(part 1 of 2)
# Autodesk Inventor assembly: ODrive Pro Assembly
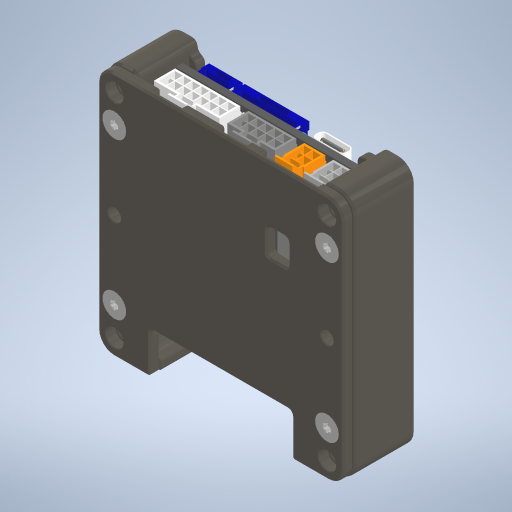
[picture p0: Inventor's stored thumbnail of the model, 512x512]
Saved by Autodesk Inventor 2023.4 (Build 274418000, 418)
## iProperties
Created: 2025-03-02
Part Number: ODrive Pro Assembly
Description: STEP AP242
Document SubType Name: Assembly
Designer: aaron
Title: 67c5018548154165ea0d0b83
Sending System: ONSHAPE BY PTC INC, 1.194
Preprocessor: ST-DEVELOPER v20
## Documents named in this file (723)
- C:\work\openworkout\digital_weight_device\cad\v5\odrive\ODrive Pro Assembly\ODrive Pro Assembly.iam
- C:\work\openworkout\digital_weight_device\cad\v5\odrive\ODrive Pro Assembly\92703A148_18-8 Stainless Steel Torx Flat Head Screws.ipt
- C:\work\openworkout\digital_weight_device\cad\v5\odrive\ODrive Pro Assembly\___________10 SIZE CODE G_7.ipt
- C:\work\openworkout\digital_weight_device\cad\v5\odrive\ODrive Pro Assembly\SOT23-5.ipt
- C:\work\openworkout\digital_weight_device\cad\v5\odrive\ODrive Pro Assembly\Extruded_55.ipt
- C:\work\openworkout\digital_weight_device\cad\v5\odrive\ODrive Pro Assembly\Open CASCADE STEP translator 6.8 23.2.1_6.ipt
- C:\work\openworkout\digital_weight_device\cad\v5\odrive\ODrive Pro Assembly\Extruded_11.ipt
- C:\work\openworkout\digital_weight_device\cad\v5\odrive\ODrive Pro Assembly\Extruded_52.ipt
- C:\work\openworkout\digital_weight_device\cad\v5\odrive\ODrive Pro Assembly\Extruded.ipt
- C:\work\openworkout\digital_weight_device\cad\v5\odrive\ODrive Pro Assembly\________10 SIZE CODE G_1.ipt
- C:\work\openworkout\digital_weight_device\cad\v5\odrive\ODrive Pro Assembly\Leader_24.ipt
- C:\work\openworkout\digital_weight_device\cad\v5\odrive\ODrive Pro Assembly\Extruded_19.ipt
- C:\work\openworkout\digital_weight_device\cad\v5\odrive\ODrive Pro Assembly\Open CASCADE STEP translator 6.8 23.2.1_2.ipt
- C:\work\openworkout\digital_weight_device\cad\v5\odrive\ODrive Pro Assembly\Open CASCADE STEP translator 6.8 23.2.1_2_1.ipt
- C:\work\openworkout\digital_weight_device\cad\v5\odrive\ODrive Pro Assembly\Extruded_16.ipt
- C:\work\openworkout\digital_weight_device\cad\v5\odrive\ODrive Pro Assembly\Cylinder_18.ipt
- C:\work\openworkout\digital_weight_device\cad\v5\odrive\ODrive Pro Assembly\Extruded_13.ipt
- C:\work\openworkout\digital_weight_device\cad\v5\odrive\ODrive Pro Assembly\Extruded_35.ipt
- C:\work\openworkout\digital_weight_device\cad\v5\odrive\ODrive Pro Assembly\Extruded_24.ipt
- C:\work\openworkout\digital_weight_device\cad\v5\odrive\ODrive Pro Assembly\Mid_Body_3.ipt
- C:\work\openworkout\digital_weight_device\cad\v5\odrive\ODrive Pro Assembly\Open CASCADE STEP translator 6.8 2.1.2.ipt
- C:\work\openworkout\digital_weight_device\cad\v5\odrive\ODrive Pro Assembly\RES 0603 (1608 metric)_21.ipt
- C:\work\openworkout\digital_weight_device\cad\v5\odrive\ODrive Pro Assembly\Extruded_10.ipt
- C:\work\openworkout\digital_weight_device\cad\v5\odrive\ODrive Pro Assembly\Extruded_42.ipt
- C:\work\openworkout\digital_weight_device\cad\v5\odrive\ODrive Pro Assembly\Leader_1.ipt
- C:\work\openworkout\digital_weight_device\cad\v5\odrive\ODrive Pro Assembly\Open CASCADE STEP translator 6.8 26.4.1_6.ipt
- C:\work\openworkout\digital_weight_device\cad\v5\odrive\ODrive Pro Assembly\Open CASCADE STEP translator 6.8 18.2.1.ipt
- C:\work\openworkout\digital_weight_device\cad\v5\odrive\ODrive Pro Assembly\FDMS86300DC rev A_7.ipt
- C:\work\openworkout\digital_weight_device\cad\v5\odrive\ODrive Pro Assembly\Extruded_21.ipt
- C:\work\openworkout\digital_weight_device\cad\v5\odrive\ODrive Pro Assembly\Mid_Body_1.ipt
- C:\work\openworkout\digital_weight_device\cad\v5\odrive\ODrive Pro Assembly\Extruded_31.ipt
- C:\work\openworkout\digital_weight_device\cad\v5\odrive\ODrive Pro Assembly\Extruded_6.ipt
- C:\work\openworkout\digital_weight_device\cad\v5\odrive\ODrive Pro Assembly\Extruded_34.ipt
- C:\work\openworkout\digital_weight_device\cad\v5\odrive\ODrive Pro Assembly\Cylinder_3.ipt
- C:\work\openworkout\digital_weight_device\cad\v5\odrive\ODrive Pro Assembly\Extruded_16_1.ipt
- C:\work\openworkout\digital_weight_device\cad\v5\odrive\ODrive Pro Assembly\Extruded_26.ipt
- C:\work\openworkout\digital_weight_device\cad\v5\odrive\ODrive Pro Assembly\Open CASCADE STEP translator 6.8 23.2.1_4.ipt
- C:\work\openworkout\digital_weight_device\cad\v5\odrive\ODrive Pro Assembly\Extruded_37.ipt
- C:\work\openworkout\digital_weight_device\cad\v5\odrive\ODrive Pro Assembly\Mark_4.ipt
- C:\work\openworkout\digital_weight_device\cad\v5\odrive\ODrive Pro Assembly\Open CASCADE STEP translator 6.8 23.2.1_11.ipt
- C:\work\openworkout\digital_weight_device\cad\v5\odrive\ODrive Pro Assembly\Mark.ipt
- C:\work\openworkout\digital_weight_device\cad\v5\odrive\ODrive Pro Assembly\Extruded_10_1.ipt
- C:\work\openworkout\digital_weight_device\cad\v5\odrive\ODrive Pro Assembly\Extruded_31_1.ipt
- C:\work\openworkout\digital_weight_device\cad\v5\odrive\ODrive Pro Assembly\Extruded_63.ipt
- C:\work\openworkout\digital_weight_device\cad\v5\odrive\ODrive Pro Assembly\Extruded_35_1.ipt
- C:\work\openworkout\digital_weight_device\cad\v5\odrive\ODrive Pro Assembly\Extruded_38.ipt
- C:\work\openworkout\digital_weight_device\cad\v5\odrive\ODrive Pro Assembly\Open CASCADE STEP translator 6.8 26.1.ipt
- C:\work\openworkout\digital_weight_device\cad\v5\odrive\ODrive Pro Assembly\Extruded_17.ipt
- C:\work\openworkout\digital_weight_device\cad\v5\odrive\ODrive Pro Assembly\Extruded_7.ipt
- C:\work\openworkout\digital_weight_device\cad\v5\odrive\ODrive Pro Assembly\Extruded_2.ipt
- C:\work\openworkout\digital_weight_device\cad\v5\odrive\ODrive Pro Assembly\Open CASCADE STEP translator 6.8 43.4.1_6.ipt
- C:\work\openworkout\digital_weight_device\cad\v5\odrive\ODrive Pro Assembly\Extruded_1.ipt
- C:\work\openworkout\digital_weight_device\cad\v5\odrive\ODrive Pro Assembly\Extruded_13_1.ipt
- C:\work\openworkout\digital_weight_device\cad\v5\odrive\ODrive Pro Assembly\Cylinder_8.ipt
- C:\work\openworkout\digital_weight_device\cad\v5\odrive\ODrive Pro Assembly\Extruded_3.ipt
- C:\work\openworkout\digital_weight_device\cad\v5\odrive\ODrive Pro Assembly\Open CASCADE STEP translator 6.8 2.1.1.ipt
- C:\work\openworkout\digital_weight_device\cad\v5\odrive\ODrive Pro Assembly\Extruded_4.ipt
- C:\work\openworkout\digital_weight_device\cad\v5\odrive\ODrive Pro Assembly\Extruded_10_2.ipt
- C:\work\openworkout\digital_weight_device\cad\v5\odrive\ODrive Pro Assembly\lead.ipt
- C:\work\openworkout\digital_weight_device\cad\v5\odrive\ODrive Pro Assembly\___________10 SIZE CODE G_4.ipt
- C:\work\openworkout\digital_weight_device\cad\v5\odrive\ODrive Pro Assembly\Extruded_2_1.ipt
- C:\work\openworkout\digital_weight_device\cad\v5\odrive\ODrive Pro Assembly\Mid_Body_3_1.ipt
- C:\work\openworkout\digital_weight_device\cad\v5\odrive\ODrive Pro Assembly\Extruded_23.ipt
- C:\work\openworkout\digital_weight_device\cad\v5\odrive\ODrive Pro Assembly\bottom.ipt
- C:\work\openworkout\digital_weight_device\cad\v5\odrive\ODrive Pro Assembly\Open CASCADE STEP translator 6.8 23.2.1_3.ipt
- C:\work\openworkout\digital_weight_device\cad\v5\odrive\ODrive Pro Assembly\Extruded_5.ipt
- C:\work\openworkout\digital_weight_device\cad\v5\odrive\ODrive Pro Assembly\NONE.ipt
- C:\work\openworkout\digital_weight_device\cad\v5\odrive\ODrive Pro Assembly\Extruded_2_2.ipt
- C:\work\openworkout\digital_weight_device\cad\v5\odrive\ODrive Pro Assembly\Open CASCADE STEP translator 6.8 2.1.1_1.ipt
- C:\work\openworkout\digital_weight_device\cad\v5\odrive\ODrive Pro Assembly\Extruded_6_1.ipt
- C:\work\openworkout\digital_weight_device\cad\v5\odrive\ODrive Pro Assembly\Mark_1.ipt
- C:\work\openworkout\digital_weight_device\cad\v5\odrive\ODrive Pro Assembly\Extruded_1_1.ipt
- C:\work\openworkout\digital_weight_device\cad\v5\odrive\ODrive Pro Assembly\Open CASCADE STEP translator 6.8 43.1.ipt
- C:\work\openworkout\digital_weight_device\cad\v5\odrive\ODrive Pro Assembly\Leader_17.ipt
- C:\work\openworkout\digital_weight_device\cad\v5\odrive\ODrive Pro Assembly\Open CASCADE STEP translator 6.8 43.4.1_13.ipt
- C:\work\openworkout\digital_weight_device\cad\v5\odrive\ODrive Pro Assembly\Extruded_8.ipt
- C:\work\openworkout\digital_weight_device\cad\v5\odrive\ODrive Pro Assembly\Leader_3.ipt
- C:\work\openworkout\digital_weight_device\cad\v5\odrive\ODrive Pro Assembly\Extruded_2_3.ipt
- C:\work\openworkout\digital_weight_device\cad\v5\odrive\ODrive Pro Assembly\Extruded_11_1.ipt
- C:\work\openworkout\digital_weight_device\cad\v5\odrive\ODrive Pro Assembly\Lead_4.ipt
- C:\work\openworkout\digital_weight_device\cad\v5\odrive\ODrive Pro Assembly\RPC2512_stp.ipt
- C:\work\openworkout\digital_weight_device\cad\v5\odrive\ODrive Pro Assembly\Mid_Body_2.ipt
- C:\work\openworkout\digital_weight_device\cad\v5\odrive\ODrive Pro Assembly\Extruded_3_1.ipt
- C:\work\openworkout\digital_weight_device\cad\v5\odrive\ODrive Pro Assembly\Cylinder_12.ipt
- C:\work\openworkout\digital_weight_device\cad\v5\odrive\ODrive Pro Assembly\Extruded_32.ipt
- C:\work\openworkout\digital_weight_device\cad\v5\odrive\ODrive Pro Assembly\Open CASCADE STEP translator 6.8 2.1.1_1_1.ipt
- C:\work\openworkout\digital_weight_device\cad\v5\odrive\ODrive Pro Assembly\Leader_10.ipt
- C:\work\openworkout\digital_weight_device\cad\v5\odrive\ODrive Pro Assembly\Extruded_9.ipt
- C:\work\openworkout\digital_weight_device\cad\v5\odrive\ODrive Pro Assembly\Open CASCADE STEP translator 7.5 6.74.2.1.ipt
- C:\work\openworkout\digital_weight_device\cad\v5\odrive\ODrive Pro Assembly\Extruded_2_4.ipt
- C:\work\openworkout\digital_weight_device\cad\v5\odrive\ODrive Pro Assembly\Cylinder_16.ipt
- C:\work\openworkout\digital_weight_device\cad\v5\odrive\ODrive Pro Assembly\Extruded_23_1.ipt
- C:\work\openworkout\digital_weight_device\cad\v5\odrive\ODrive Pro Assembly\Extruded_13_2.ipt
- C:\work\openworkout\digital_weight_device\cad\v5\odrive\ODrive Pro Assembly\Extruded_12.ipt
- C:\work\openworkout\digital_weight_device\cad\v5\odrive\ODrive Pro Assembly\________10 SIZE CODE G.ipt
- C:\work\openworkout\digital_weight_device\cad\v5\odrive\ODrive Pro Assembly\Leader_23.ipt
- C:\work\openworkout\digital_weight_device\cad\v5\odrive\ODrive Pro Assembly\Extruded_18.ipt
- C:\work\openworkout\digital_weight_device\cad\v5\odrive\ODrive Pro Assembly\Mid_Body_1_1.ipt
- C:\work\openworkout\digital_weight_device\cad\v5\odrive\ODrive Pro Assembly\Mid_Body_1_2.ipt
- C:\work\openworkout\digital_weight_device\cad\v5\odrive\ODrive Pro Assembly\Extruded_7_1.ipt
- C:\work\openworkout\digital_weight_device\cad\v5\odrive\ODrive Pro Assembly\Extruded_22.ipt
- C:\work\openworkout\digital_weight_device\cad\v5\odrive\ODrive Pro Assembly\Extruded_12_1.ipt
- C:\work\openworkout\digital_weight_device\cad\v5\odrive\ODrive Pro Assembly\Extruded_34_1.ipt
- C:\work\openworkout\digital_weight_device\cad\v5\odrive\ODrive Pro Assembly\Extruded_49.ipt
- C:\work\openworkout\digital_weight_device\cad\v5\odrive\ODrive Pro Assembly\Mark_2.ipt
- C:\work\openworkout\digital_weight_device\cad\v5\odrive\ODrive Pro Assembly\Open CASCADE STEP translator 6.8 2.1.1_2.ipt
- C:\work\openworkout\digital_weight_device\cad\v5\odrive\ODrive Pro Assembly\RES 0603 (1608 metric)_20.ipt
- C:\work\openworkout\digital_weight_device\cad\v5\odrive\ODrive Pro Assembly\Extruded_3_2.ipt
- C:\work\openworkout\digital_weight_device\cad\v5\odrive\ODrive Pro Assembly\Extruded_7_2.ipt
- C:\work\openworkout\digital_weight_device\cad\v5\odrive\ODrive Pro Assembly\Leader.ipt
- C:\work\openworkout\digital_weight_device\cad\v5\odrive\ODrive Pro Assembly\Open CASCADE STEP translator 6.8 26.4.1_5.ipt
- C:\work\openworkout\digital_weight_device\cad\v5\odrive\ODrive Pro Assembly\Mid_Body.ipt
- C:\work\openworkout\digital_weight_device\cad\v5\odrive\ODrive Pro Assembly\FDMS86300DC rev A_6.ipt
- C:\work\openworkout\digital_weight_device\cad\v5\odrive\ODrive Pro Assembly\Extruded_43.ipt
- C:\work\openworkout\digital_weight_device\cad\v5\odrive\ODrive Pro Assembly\Mark_3.ipt
- C:\work\openworkout\digital_weight_device\cad\v5\odrive\ODrive Pro Assembly\Extruded_15.ipt
- C:\work\openworkout\digital_weight_device\cad\v5\odrive\ODrive Pro Assembly\Extruded_13_3.ipt
- C:\work\openworkout\digital_weight_device\cad\v5\odrive\ODrive Pro Assembly\RES 0603 (1608 metric)_11.ipt
- C:\work\openworkout\digital_weight_device\cad\v5\odrive\ODrive Pro Assembly\Cylinder_2.ipt
- C:\work\openworkout\digital_weight_device\cad\v5\odrive\ODrive Pro Assembly\Extruded_33.ipt
- C:\work\openworkout\digital_weight_device\cad\v5\odrive\ODrive Pro Assembly\Extruded_12_2.ipt
- C:\work\openworkout\digital_weight_device\cad\v5\odrive\ODrive Pro Assembly\Mid_Body_2_1.ipt
- C:\work\openworkout\digital_weight_device\cad\v5\odrive\ODrive Pro Assembly\Extruded_36.ipt
- C:\work\openworkout\digital_weight_device\cad\v5\odrive\ODrive Pro Assembly\Extruded_9_1.ipt
- C:\work\openworkout\digital_weight_device\cad\v5\odrive\ODrive Pro Assembly\Open CASCADE STEP translator 6.8 2.1.1_3.ipt
- C:\work\openworkout\digital_weight_device\cad\v5\odrive\ODrive Pro Assembly\______10 SIZE CODE G_2.ipt
- C:\work\openworkout\digital_weight_device\cad\v5\odrive\ODrive Pro Assembly\Extruded_5_1.ipt
- C:\work\openworkout\digital_weight_device\cad\v5\odrive\ODrive Pro Assembly\Extruded_12_3.ipt
- C:\work\openworkout\digital_weight_device\cad\v5\odrive\ODrive Pro Assembly\Open CASCADE STEP translator 6.8 23.2.1_9.ipt
- C:\work\openworkout\digital_weight_device\cad\v5\odrive\ODrive Pro Assembly\Open CASCADE STEP translator 6.8 23.2.1_10.ipt
- C:\work\openworkout\digital_weight_device\cad\v5\odrive\ODrive Pro Assembly\Open CASCADE STEP translator 6.8 1.2.1_1.ipt
- C:\work\openworkout\digital_weight_device\cad\v5\odrive\ODrive Pro Assembly\Extruded_19_1.ipt
- C:\work\openworkout\digital_weight_device\cad\v5\odrive\ODrive Pro Assembly\Extruded_30.ipt
- C:\work\openworkout\digital_weight_device\cad\v5\odrive\ODrive Pro Assembly\Extruded_62.ipt
- C:\work\openworkout\digital_weight_device\cad\v5\odrive\ODrive Pro Assembly\Extruded_34_2.ipt
- C:\work\openworkout\digital_weight_device\cad\v5\odrive\ODrive Pro Assembly\Mark_4_1.ipt
- C:\work\openworkout\digital_weight_device\cad\v5\odrive\ODrive Pro Assembly\Extruded_20.ipt
- C:\work\openworkout\digital_weight_device\cad\v5\odrive\ODrive Pro Assembly\Extruded_16_2.ipt
- C:\work\openworkout\digital_weight_device\cad\v5\odrive\ODrive Pro Assembly\___________10 SIZE CODE G_6.ipt
- C:\work\openworkout\digital_weight_device\cad\v5\odrive\ODrive Pro Assembly\Extruded_12_4.ipt
- C:\work\openworkout\digital_weight_device\cad\v5\odrive\ODrive Pro Assembly\Extruded_54.ipt
- C:\work\openworkout\digital_weight_device\cad\v5\odrive\ODrive Pro Assembly\Mid_Body_3_2.ipt
- C:\work\openworkout\digital_weight_device\cad\v5\odrive\ODrive Pro Assembly\Open CASCADE STEP translator 6.8 43.4.1_5.ipt
- C:\work\openworkout\digital_weight_device\cad\v5\odrive\ODrive Pro Assembly\Extruded_3_3.ipt
- C:\work\openworkout\digital_weight_device\cad\v5\odrive\ODrive Pro Assembly\Extruded_12_5.ipt
- C:\work\openworkout\digital_weight_device\cad\v5\odrive\ODrive Pro Assembly\Cylinder_7.ipt
- C:\work\openworkout\digital_weight_device\cad\v5\odrive\ODrive Pro Assembly\Extruded_1_2.ipt
- C:\work\openworkout\digital_weight_device\cad\v5\odrive\ODrive Pro Assembly\Open CASCADE STEP translator 6.8 19.2.1.ipt
- C:\work\openworkout\digital_weight_device\cad\v5\odrive\ODrive Pro Assembly\Extruded_1_3.ipt
- C:\work\openworkout\digital_weight_device\cad\v5\odrive\ODrive Pro Assembly\Extruded_22_1.ipt
- C:\work\openworkout\digital_weight_device\cad\v5\odrive\ODrive Pro Assembly\top.ipt
- C:\work\openworkout\digital_weight_device\cad\v5\odrive\ODrive Pro Assembly\Open CASCADE STEP translator 6.8 23.2.1_2_2.ipt
- C:\work\openworkout\digital_weight_device\cad\v5\odrive\ODrive Pro Assembly\Extruded_7_3.ipt
- C:\work\openworkout\digital_weight_device\cad\v5\odrive\ODrive Pro Assembly\Cylinder_9.ipt
- C:\work\openworkout\digital_weight_device\cad\v5\odrive\ODrive Pro Assembly\SM05B-GHS-TB.ipt
- C:\work\openworkout\digital_weight_device\cad\v5\odrive\ODrive Pro Assembly\Mark_2_1.ipt
- C:\work\openworkout\digital_weight_device\cad\v5\odrive\ODrive Pro Assembly\Extruded_5_2.ipt
- C:\work\openworkout\digital_weight_device\cad\v5\odrive\ODrive Pro Assembly\Open CASCADE STEP translator 6.8 23.2.1_1.ipt
- C:\work\openworkout\digital_weight_device\cad\v5\odrive\ODrive Pro Assembly\Extruded_14.ipt
- C:\work\openworkout\digital_weight_device\cad\v5\odrive\ODrive Pro Assembly\Extruded_4_1.ipt
- C:\work\openworkout\digital_weight_device\cad\v5\odrive\ODrive Pro Assembly\Leader_16.ipt
- C:\work\openworkout\digital_weight_device\cad\v5\odrive\ODrive Pro Assembly\Open CASCADE STEP translator 6.8 43.4.1_12.ipt
- C:\work\openworkout\digital_weight_device\cad\v5\odrive\ODrive Pro Assembly\Extruded_16_3.ipt
- C:\work\openworkout\digital_weight_device\cad\v5\odrive\ODrive Pro Assembly\Leader_2.ipt
- C:\work\openworkout\digital_weight_device\cad\v5\odrive\ODrive Pro Assembly\Extruded_25.ipt
- C:\work\openworkout\digital_weight_device\cad\v5\odrive\ODrive Pro Assembly\Extruded_5_3.ipt
- C:\work\openworkout\digital_weight_device\cad\v5\odrive\ODrive Pro Assembly\Lead_3.ipt
- C:\work\openworkout\digital_weight_device\cad\v5\odrive\ODrive Pro Assembly\RPC2512_stp_1.ipt
- C:\work\openworkout\digital_weight_device\cad\v5\odrive\ODrive Pro Assembly\Mark_1_1.ipt
- C:\work\openworkout\digital_weight_device\cad\v5\odrive\ODrive Pro Assembly\Extruded_6_2.ipt
- C:\work\openworkout\digital_weight_device\cad\v5\odrive\ODrive Pro Assembly\Cylinder_11.ipt
- C:\work\openworkout\digital_weight_device\cad\v5\odrive\ODrive Pro Assembly\Extruded_15_1.ipt
- C:\work\openworkout\digital_weight_device\cad\v5\odrive\ODrive Pro Assembly\Leader_2_1.ipt
- C:\work\openworkout\digital_weight_device\cad\v5\odrive\ODrive Pro Assembly\Leader_9.ipt
- C:\work\openworkout\digital_weight_device\cad\v5\odrive\ODrive Pro Assembly\Extruded_19_2.ipt
- C:\work\openworkout\digital_weight_device\cad\v5\odrive\ODrive Pro Assembly\Extruded_5_4.ipt
- C:\work\openworkout\digital_weight_device\cad\v5\odrive\ODrive Pro Assembly\Cylinder_15.ipt
- C:\work\openworkout\digital_weight_device\cad\v5\odrive\ODrive Pro Assembly\Extruded_15_2.ipt
- C:\work\openworkout\digital_weight_device\cad\v5\odrive\ODrive Pro Assembly\Extruded_5_5.ipt
- C:\work\openworkout\digital_weight_device\cad\v5\odrive\ODrive Pro Assembly\Leader_22.ipt
- C:\work\openworkout\digital_weight_device\cad\v5\odrive\ODrive Pro Assembly\Extruded_27.ipt
- C:\work\openworkout\digital_weight_device\cad\v5\odrive\ODrive Pro Assembly\Extruded_9_2.ipt
- C:\work\openworkout\digital_weight_device\cad\v5\odrive\ODrive Pro Assembly\Mark_5.ipt
- C:\work\openworkout\digital_weight_device\cad\v5\odrive\ODrive Pro Assembly\Extruded_15_3.ipt
- C:\work\openworkout\digital_weight_device\cad\v5\odrive\ODrive Pro Assembly\Extruded_48.ipt
- C:\work\openworkout\digital_weight_device\cad\v5\odrive\ODrive Pro Assembly\Open CASCADE STEP translator 6.8 2.2.1_2.ipt
- C:\work\openworkout\digital_weight_device\cad\v5\odrive\ODrive Pro Assembly\Extruded_3_4.ipt
- C:\work\openworkout\digital_weight_device\cad\v5\odrive\ODrive Pro Assembly\Open CASCADE STEP translator 6.8 5.2.1.ipt
- C:\work\openworkout\digital_weight_device\cad\v5\odrive\ODrive Pro Assembly\Leader_15.ipt
- C:\work\openworkout\digital_weight_device\cad\v5\odrive\ODrive Pro Assembly\Extruded_42_1.ipt
- C:\work\openworkout\digital_weight_device\cad\v5\odrive\ODrive Pro Assembly\Open CASCADE STEP translator 7.5 6.122.1.1.ipt
- C:\work\openworkout\digital_weight_device\cad\v5\odrive\ODrive Pro Assembly\Extruded_12_6.ipt
- C:\work\openworkout\digital_weight_device\cad\v5\odrive\ODrive Pro Assembly\Cylinder_1.ipt
- C:\work\openworkout\digital_weight_device\cad\v5\odrive\ODrive Pro Assembly\Extruded_25_1.ipt
- C:\work\openworkout\digital_weight_device\cad\v5\odrive\ODrive Pro Assembly\Extruded_17_1.ipt
- C:\work\openworkout\digital_weight_device\cad\v5\odrive\ODrive Pro Assembly\Extruded_4_2.ipt
- C:\work\openworkout\digital_weight_device\cad\v5\odrive\ODrive Pro Assembly\Open CASCADE STEP translator 6.8 2.1.1_4.ipt
- C:\work\openworkout\digital_weight_device\cad\v5\odrive\ODrive Pro Assembly\Extruded_3_5.ipt
- C:\work\openworkout\digital_weight_device\cad\v5\odrive\ODrive Pro Assembly\TSSOP65P640X120-16N.ipt
- C:\work\openworkout\digital_weight_device\cad\v5\odrive\ODrive Pro Assembly\Extruded_11_2.ipt
- C:\work\openworkout\digital_weight_device\cad\v5\odrive\ODrive Pro Assembly\Open CASCADE STEP translator 6.8 23.2.1_8.ipt
- C:\work\openworkout\digital_weight_device\cad\v5\odrive\ODrive Pro Assembly\Mid_Body_5.ipt
- C:\work\openworkout\digital_weight_device\cad\v5\odrive\ODrive Pro Assembly\Open CASCADE STEP translator 6.8 1.2.1.ipt
- C:\work\openworkout\digital_weight_device\cad\v5\odrive\ODrive Pro Assembly\Extruded_18_1.ipt
- C:\work\openworkout\digital_weight_device\cad\v5\odrive\ODrive Pro Assembly\Extruded_14_1.ipt
- C:\work\openworkout\digital_weight_device\cad\v5\odrive\ODrive Pro Assembly\Extruded_30_1.ipt
- C:\work\openworkout\digital_weight_device\cad\v5\odrive\ODrive Pro Assembly\RES 0603 (1608 metric)_13.ipt
- C:\work\openworkout\digital_weight_device\cad\v5\odrive\ODrive Pro Assembly\Open CASCADE STEP translator 6.8 23.2.1_9_1.ipt
- C:\work\openworkout\digital_weight_device\cad\v5\odrive\ODrive Pro Assembly\Extruded_41.ipt
- C:\work\openworkout\digital_weight_device\cad\v5\odrive\ODrive Pro Assembly\RES 0603 (1608 metric)_15.ipt
- C:\work\openworkout\digital_weight_device\cad\v5\odrive\ODrive Pro Assembly\______10 SIZE CODE G_3.ipt
- C:\work\openworkout\digital_weight_device\cad\v5\odrive\ODrive Pro Assembly\Extruded_25_2.ipt
- C:\work\openworkout\digital_weight_device\cad\v5\odrive\ODrive Pro Assembly\Extruded_28.ipt
- C:\work\openworkout\digital_weight_device\cad\v5\odrive\ODrive Pro Assembly\Extruded_15_4.ipt
- C:\work\openworkout\digital_weight_device\cad\v5\odrive\ODrive Pro Assembly\Extruded_22_2.ipt
- C:\work\openworkout\digital_weight_device\cad\v5\odrive\ODrive Pro Assembly\Extruded_12_7.ipt
- C:\work\openworkout\digital_weight_device\cad\v5\odrive\ODrive Pro Assembly\Extruded_13_4.ipt
- C:\work\openworkout\digital_weight_device\cad\v5\odrive\ODrive Pro Assembly\___________10 SIZE CODE G_1.ipt
- C:\work\openworkout\digital_weight_device\cad\v5\odrive\ODrive Pro Assembly\Extruded_29.ipt
- C:\work\openworkout\digital_weight_device\cad\v5\odrive\ODrive Pro Assembly\Extruded_39.ipt
- C:\work\openworkout\digital_weight_device\cad\v5\odrive\ODrive Pro Assembly\Cylinder_6.ipt
- C:\work\openworkout\digital_weight_device\cad\v5\odrive\ODrive Pro Assembly\Cylinder_5.ipt
- C:\work\openworkout\digital_weight_device\cad\v5\odrive\ODrive Pro Assembly\Cylinder_4.ipt
- C:\work\openworkout\digital_weight_device\cad\v5\odrive\ODrive Pro Assembly\Cylinder_3_1.ipt
- C:\work\openworkout\digital_weight_device\cad\v5\odrive\ODrive Pro Assembly\Cylinder_2_1.ipt
- C:\work\openworkout\digital_weight_device\cad\v5\odrive\ODrive Pro Assembly\Extruded_40.ipt
- C:\work\openworkout\digital_weight_device\cad\v5\odrive\ODrive Pro Assembly\Extruded_9_3.ipt
- C:\work\openworkout\digital_weight_device\cad\v5\odrive\ODrive Pro Assembly\Open CASCADE STEP translator 6.8 43.4.1_11.ipt
- C:\work\openworkout\digital_weight_device\cad\v5\odrive\ODrive Pro Assembly\Cylinder_1_1.ipt
- C:\work\openworkout\digital_weight_device\cad\v5\odrive\ODrive Pro Assembly\Leader_1_1.ipt
- C:\work\openworkout\digital_weight_device\cad\v5\odrive\ODrive Pro Assembly\Cylinder.ipt
- C:\work\openworkout\digital_weight_device\cad\v5\odrive\ODrive Pro Assembly\Extruded_1_4.ipt
- C:\work\openworkout\digital_weight_device\cad\v5\odrive\ODrive Pro Assembly\Cylinder_2_2.ipt
- C:\work\openworkout\digital_weight_device\cad\v5\odrive\ODrive Pro Assembly\Cylinder_1_2.ipt
- C:\work\openworkout\digital_weight_device\cad\v5\odrive\ODrive Pro Assembly\Cylinder_10.ipt
- C:\work\openworkout\digital_weight_device\cad\v5\odrive\ODrive Pro Assembly\Open CASCADE STEP translator 7.5 6.1.1.ipt
- C:\work\openworkout\digital_weight_device\cad\v5\odrive\ODrive Pro Assembly\RES 0603 (1608 metric).ipt
- C:\work\openworkout\digital_weight_device\cad\v5\odrive\ODrive Pro Assembly\Extruded_1_5.ipt
- C:\work\openworkout\digital_weight_device\cad\v5\odrive\ODrive Pro Assembly\Extruded_44.ipt
- C:\work\openworkout\digital_weight_device\cad\v5\odrive\ODrive Pro Assembly\RES 0603 (1608 metric)_16.ipt
- C:\work\openworkout\digital_weight_device\cad\v5\odrive\ODrive Pro Assembly\Open CASCADE STEP translator 6.8 23.2.1_13.ipt
- C:\work\openworkout\digital_weight_device\cad\v5\odrive\ODrive Pro Assembly\Mark_1_2.ipt
- C:\work\openworkout\digital_weight_device\cad\v5\odrive\ODrive Pro Assembly\Extruded_23_2.ipt
- C:\work\openworkout\digital_weight_device\cad\v5\odrive\ODrive Pro Assembly\Extruded_29_1.ipt
- C:\work\openworkout\digital_weight_device\cad\v5\odrive\ODrive Pro Assembly\Extruded_32_1.ipt
- C:\work\openworkout\digital_weight_device\cad\v5\odrive\ODrive Pro Assembly\Extruded_19_3.ipt
- C:\work\openworkout\digital_weight_device\cad\v5\odrive\ODrive Pro Assembly\Extruded_41_1.ipt
- C:\work\openworkout\digital_weight_device\cad\v5\odrive\ODrive Pro Assembly\Open CASCADE STEP translator 6.8 26.4.1_1.ipt
- C:\work\openworkout\digital_weight_device\cad\v5\odrive\ODrive Pro Assembly\FDMS86300DC rev A_2.ipt
- C:\work\openworkout\digital_weight_device\cad\v5\odrive\ODrive Pro Assembly\Extruded_15_5.ipt
- C:\work\openworkout\digital_weight_device\cad\v5\odrive\ODrive Pro Assembly\Extruded_28_1.ipt
- C:\work\openworkout\digital_weight_device\cad\v5\odrive\ODrive Pro Assembly\Extruded_14_2.ipt
- C:\work\openworkout\digital_weight_device\cad\v5\odrive\ODrive Pro Assembly\Open CASCADE STEP translator 6.8 23.2.1_8_1.ipt
- C:\work\openworkout\digital_weight_device\cad\v5\odrive\ODrive Pro Assembly\Mark_2_2.ipt
- C:\work\openworkout\digital_weight_device\cad\v5\odrive\ODrive Pro Assembly\Extruded_13_5.ipt
- C:\work\openworkout\digital_weight_device\cad\v5\odrive\ODrive Pro Assembly\Extruded_15_6.ipt
- C:\work\openworkout\digital_weight_device\cad\v5\odrive\ODrive Pro Assembly\___________10 SIZE CODE G_3.ipt
- C:\work\openworkout\digital_weight_device\cad\v5\odrive\ODrive Pro Assembly\Leader_28.ipt
- C:\work\openworkout\digital_weight_device\cad\v5\odrive\ODrive Pro Assembly\Extruded_21_1.ipt
- C:\work\openworkout\digital_weight_device\cad\v5\odrive\ODrive Pro Assembly\Open CASCADE STEP translator 6.8 23.2.1.ipt
- C:\work\openworkout\digital_weight_device\cad\v5\odrive\ODrive Pro Assembly\Extruded_11_3.ipt
- C:\work\openworkout\digital_weight_device\cad\v5\odrive\ODrive Pro Assembly\Extruded_7_4.ipt
- C:\work\openworkout\digital_weight_device\cad\v5\odrive\ODrive Pro Assembly\Open CASCADE STEP translator 6.8 2.1.2_2.ipt
- C:\work\openworkout\digital_weight_device\cad\v5\odrive\ODrive Pro Assembly\Extruded_9_4.ipt
- C:\work\openworkout\digital_weight_device\cad\v5\odrive\ODrive Pro Assembly\Extruded_1_6.ipt
- C:\work\openworkout\digital_weight_device\cad\v5\odrive\ODrive Pro Assembly\Lead_1.ipt
- C:\work\openworkout\digital_weight_device\cad\v5\odrive\ODrive Pro Assembly\Mid_Body_4.ipt
- C:\work\openworkout\digital_weight_device\cad\v5\odrive\ODrive Pro Assembly\Extruded_20_1.ipt
- C:\work\openworkout\digital_weight_device\cad\v5\odrive\ODrive Pro Assembly\Mark_6.ipt
- C:\work\openworkout\digital_weight_device\cad\v5\odrive\ODrive Pro Assembly\SM12B-GHS-TB.ipt
- C:\work\openworkout\digital_weight_device\cad\v5\odrive\ODrive Pro Assembly\Open CASCADE STEP translator 6.8 23.2.1_2_3.ipt
- C:\work\openworkout\digital_weight_device\cad\v5\odrive\ODrive Pro Assembly\Extruded_23_3.ipt
- C:\work\openworkout\digital_weight_device\cad\v5\odrive\ODrive Pro Assembly\Extruded_24_1.ipt
- C:\work\openworkout\digital_weight_device\cad\v5\odrive\ODrive Pro Assembly\Cylinder_9_1.ipt
- C:\work\openworkout\digital_weight_device\cad\v5\odrive\ODrive Pro Assembly\Extruded_35_2.ipt
- C:\work\openworkout\digital_weight_device\cad\v5\odrive\ODrive Pro Assembly\Extruded_30_2.ipt
- C:\work\openworkout\digital_weight_device\cad\v5\odrive\ODrive Pro Assembly\Open CASCADE STEP translator 6.8 5.1.ipt
- C:\work\openworkout\digital_weight_device\cad\v5\odrive\ODrive Pro Assembly\Leader_4.ipt
- C:\work\openworkout\digital_weight_device\cad\v5\odrive\ODrive Pro Assembly\Leader_14.ipt
- C:\work\openworkout\digital_weight_device\cad\v5\odrive\ODrive Pro Assembly\Leader_7.ipt
- C:\work\openworkout\digital_weight_device\cad\v5\odrive\ODrive Pro Assembly\Extruded_10_3.ipt
- C:\work\openworkout\digital_weight_device\cad\v5\odrive\ODrive Pro Assembly\RES 0603 (1608 metric)_2.ipt
- C:\work\openworkout\digital_weight_device\cad\v5\odrive\ODrive Pro Assembly\Extruded_4_3.ipt
- C:\work\openworkout\digital_weight_device\cad\v5\odrive\ODrive Pro Assembly\Open CASCADE STEP translator 6.8 2.2.1.ipt
- C:\work\openworkout\digital_weight_device\cad\v5\odrive\ODrive Pro Assembly\Extruded_45.ipt
- C:\work\openworkout\digital_weight_device\cad\v5\odrive\ODrive Pro Assembly\Extruded_4_4.ipt
- C:\work\openworkout\digital_weight_device\cad\v5\odrive\ODrive Pro Assembly\Cylinder_13.ipt
- C:\work\openworkout\digital_weight_device\cad\v5\odrive\ODrive Pro Assembly\Cylinder_3_2.ipt
- C:\work\openworkout\digital_weight_device\cad\v5\odrive\ODrive Pro Assembly\Extruded_3_6.ipt
- C:\work\openworkout\digital_weight_device\cad\v5\odrive\ODrive Pro Assembly\Extruded_10_4.ipt
- C:\work\openworkout\digital_weight_device\cad\v5\odrive\ODrive Pro Assembly\Open CASCADE STEP translator 6.8 2.2.1_1.ipt
- C:\work\openworkout\digital_weight_device\cad\v5\odrive\ODrive Pro Assembly\Open CASCADE STEP translator 6.8 43.4.1_10.ipt
- C:\work\openworkout\digital_weight_device\cad\v5\odrive\ODrive Pro Assembly\Open CASCADE STEP translator 6.8 43.4.1_3.ipt
- C:\work\openworkout\digital_weight_device\cad\v5\odrive\ODrive Pro Assembly\Leader_5.ipt
- C:\work\openworkout\digital_weight_device\cad\v5\odrive\ODrive Pro Assembly\Extruded_5_6.ipt
- C:\work\openworkout\digital_weight_device\cad\v5\odrive\ODrive Pro Assembly\Extruded_1_7.ipt
- C:\work\openworkout\digital_weight_device\cad\v5\odrive\ODrive Pro Assembly\Extruded_3_7.ipt
- C:\work\openworkout\digital_weight_device\cad\v5\odrive\ODrive Pro Assembly\Extruded_6_3.ipt
- C:\work\openworkout\digital_weight_device\cad\v5\odrive\ODrive Pro Assembly\Extruded_1_8.ipt
- C:\work\openworkout\digital_weight_device\cad\v5\odrive\ODrive Pro Assembly\Extruded_46.ipt
- C:\work\openworkout\digital_weight_device\cad\v5\odrive\ODrive Pro Assembly\Extruded_47.ipt
- C:\work\openworkout\digital_weight_device\cad\v5\odrive\ODrive Pro Assembly\Open CASCADE STEP translator 6.8 19.1.1.ipt
- C:\work\openworkout\digital_weight_device\cad\v5\odrive\ODrive Pro Assembly\Extruded_8_1.ipt
- C:\work\openworkout\digital_weight_device\cad\v5\odrive\ODrive Pro Assembly\Extruded_3_8.ipt
- C:\work\openworkout\digital_weight_device\cad\v5\odrive\ODrive Pro Assembly\Extruded_44_1.ipt
- C:\work\openworkout\digital_weight_device\cad\v5\odrive\ODrive Pro Assembly\Extruded_29_2.ipt
- C:\work\openworkout\digital_weight_device\cad\v5\odrive\ODrive Pro Assembly\Extruded_24_2.ipt
- C:\work\openworkout\digital_weight_device\cad\v5\odrive\ODrive Pro Assembly\Extruded_61.ipt
- C:\work\openworkout\digital_weight_device\cad\v5\odrive\ODrive Pro Assembly\Extruded_33_1.ipt
- C:\work\openworkout\digital_weight_device\cad\v5\odrive\ODrive Pro Assembly\Extruded_8_2.ipt
- C:\work\openworkout\digital_weight_device\cad\v5\odrive\ODrive Pro Assembly\Mid_Body_4_1.ipt
- C:\work\openworkout\digital_weight_device\cad\v5\odrive\ODrive Pro Assembly\Open CASCADE STEP translator 6.8 1.2.1_4.ipt
- C:\work\openworkout\digital_weight_device\cad\v5\odrive\ODrive Pro Assembly\Open CASCADE STEP translator 6.8 8.2.1.ipt
- C:\work\openworkout\digital_weight_device\cad\v5\odrive\ODrive Pro Assembly\Mark_3_1.ipt
- C:\work\openworkout\digital_weight_device\cad\v5\odrive\ODrive Pro Assembly\RES 0603 (1608 metric)_18.ipt
- C:\work\openworkout\digital_weight_device\cad\v5\odrive\ODrive Pro Assembly\RES 0603 (1608 metric)_7.ipt
- C:\work\openworkout\digital_weight_device\cad\v5\odrive\ODrive Pro Assembly\Extruded_40_1.ipt
- C:\work\openworkout\digital_weight_device\cad\v5\odrive\ODrive Pro Assembly\Extruded_14_3.ipt
- C:\work\openworkout\digital_weight_device\cad\v5\odrive\ODrive Pro Assembly\Leader_5_1.ipt
- C:\work\openworkout\digital_weight_device\cad\v5\odrive\ODrive Pro Assembly\Extruded_28_2.ipt
- C:\work\openworkout\digital_weight_device\cad\v5\odrive\ODrive Pro Assembly\Open CASCADE STEP translator 6.8 26.4.1_3.ipt
- C:\work\openworkout\digital_weight_device\cad\v5\odrive\ODrive Pro Assembly\Open CASCADE STEP translator 6.8 18.2.1_1.ipt
- C:\work\openworkout\digital_weight_device\cad\v5\odrive\ODrive Pro Assembly\Mid_Body_6.ipt
- C:\work\openworkout\digital_weight_device\cad\v5\odrive\ODrive Pro Assembly\FDMS86300DC rev A_4.ipt
- C:\work\openworkout\digital_weight_device\cad\v5\odrive\ODrive Pro Assembly\RES 0603 (1608 metric)_5.ipt
- C:\work\openworkout\digital_weight_device\cad\v5\odrive\ODrive Pro Assembly\Extruded_9_5.ipt
- C:\work\openworkout\digital_weight_device\cad\v5\odrive\ODrive Pro Assembly\Open CASCADE STEP translator 6.8 1.2.1_2.ipt
- C:\work\openworkout\digital_weight_device\cad\v5\odrive\ODrive Pro Assembly\Extruded_50.ipt
- C:\work\openworkout\digital_weight_device\cad\v5\odrive\ODrive Pro Assembly\Extruded_14_4.ipt
- C:\work\openworkout\digital_weight_device\cad\v5\odrive\ODrive Pro Assembly\Mark_7.ipt
- C:\work\openworkout\digital_weight_device\cad\v5\odrive\ODrive Pro Assembly\Extruded_31_2.ipt
- C:\work\openworkout\digital_weight_device\cad\v5\odrive\ODrive Pro Assembly\Extruded_33_2.ipt
- C:\work\openworkout\digital_weight_device\cad\v5\odrive\ODrive Pro Assembly\Cylinder_7_1.ipt
- C:\work\openworkout\digital_weight_device\cad\v5\odrive\ODrive Pro Assembly\RES 0603 (1608 metric)_12.ipt
- C:\work\openworkout\digital_weight_device\cad\v5\odrive\ODrive Pro Assembly\Mark_4_2.ipt
- C:\work\openworkout\digital_weight_device\cad\v5\odrive\ODrive Pro Assembly\Extruded_29_3.ipt
- C:\work\openworkout\digital_weight_device\cad\v5\odrive\ODrive Pro Assembly\Open CASCADE STEP translator 6.8 23.2.1_8_2.ipt
- C:\work\openworkout\digital_weight_device\cad\v5\odrive\ODrive Pro Assembly\Extruded_37_1.ipt
- C:\work\openworkout\digital_weight_device\cad\v5\odrive\ODrive Pro Assembly\Extruded_19_4.ipt
- C:\work\openworkout\digital_weight_device\cad\v5\odrive\ODrive Pro Assembly\Extruded_6_4.ipt
- C:\work\openworkout\digital_weight_device\cad\v5\odrive\ODrive Pro Assembly\Extruded_8_3.ipt
- C:\work\openworkout\digital_weight_device\cad\v5\odrive\ODrive Pro Assembly\___________10 SIZE CODE G.ipt
- C:\work\openworkout\digital_weight_device\cad\v5\odrive\ODrive Pro Assembly\Extruded_8_4.ipt
- C:\work\openworkout\digital_weight_device\cad\v5\odrive\ODrive Pro Assembly\_______10x9.5L SIDE CODE G_3.ipt
- C:\work\openworkout\digital_weight_device\cad\v5\odrive\ODrive Pro Assembly\________10 SIZE CODE G_3.ipt
- C:\work\openworkout\digital_weight_device\cad\v5\odrive\ODrive Pro Assembly\Extruded_8_5.ipt
- C:\work\openworkout\digital_weight_device\cad\v5\odrive\ODrive Pro Assembly\Extruded_24_3.ipt
- C:\work\openworkout\digital_weight_device\cad\v5\odrive\ODrive Pro Assembly\Extruded_24_4.ipt
- C:\work\openworkout\digital_weight_device\cad\v5\odrive\ODrive Pro Assembly\Extruded_19_5.ipt
- C:\work\openworkout\digital_weight_device\cad\v5\odrive\ODrive Pro Assembly\Extruded_1_9.ipt
- C:\work\openworkout\digital_weight_device\cad\v5\odrive\ODrive Pro Assembly\Open CASCADE STEP translator 6.8 23.2.1_1_1.ipt
- C:\work\openworkout\digital_weight_device\cad\v5\odrive\ODrive Pro Assembly\Mark_8.ipt
- C:\work\openworkout\digital_weight_device\cad\v5\odrive\ODrive Pro Assembly\Extruded_6_5.ipt
- C:\work\openworkout\digital_weight_device\cad\v5\odrive\ODrive Pro Assembly\Extruded_10_5.ipt
- C:\work\openworkout\digital_weight_device\cad\v5\odrive\ODrive Pro Assembly\Cylinder_7_2.ipt
- C:\work\openworkout\digital_weight_device\cad\v5\odrive\ODrive Pro Assembly\Open CASCADE STEP translator 6.8 2.1.1_5.ipt
- C:\work\openworkout\digital_weight_device\cad\v5\odrive\ODrive Pro Assembly\Extruded_6_6.ipt
- C:\work\openworkout\digital_weight_device\cad\v5\odrive\ODrive Pro Assembly\Open CASCADE STEP translator 6.8 23.2.1_4_1.ipt
- C:\work\openworkout\digital_weight_device\cad\v5\odrive\ODrive Pro Assembly\Open CASCADE STEP translator 7.5 6.74.2.1_1.ipt
- C:\work\openworkout\digital_weight_device\cad\v5\odrive\ODrive Pro Assembly\Extruded_6_7.ipt
- C:\work\openworkout\digital_weight_device\cad\v5\odrive\ODrive Pro Assembly\Extruded_14_5.ipt
- C:\work\openworkout\digital_weight_device\cad\v5\odrive\ODrive Pro Assembly\Open CASCADE STEP translator 6.8 43.4.1_1.ipt
- C:\work\openworkout\digital_weight_device\cad\v5\odrive\ODrive Pro Assembly\Leader_21.ipt
- C:\work\openworkout\digital_weight_device\cad\v5\odrive\ODrive Pro Assembly\Open CASCADE STEP translator 6.8 5.1_1.ipt
- C:\work\openworkout\digital_weight_device\cad\v5\odrive\ODrive Pro Assembly\Extruded_10_6.ipt
- C:\work\openworkout\digital_weight_device\cad\v5\odrive\ODrive Pro Assembly\Extruded_51.ipt
- C:\work\openworkout\digital_weight_device\cad\v5\odrive\ODrive Pro Assembly\Leader_30.ipt
- C:\work\openworkout\digital_weight_device\cad\v5\odrive\ODrive Pro Assembly\Leader_7_1.ipt
- C:\work\openworkout\digital_weight_device\cad\v5\odrive\ODrive Pro Assembly\Extruded_5_7.ipt
- C:\work\openworkout\digital_weight_device\cad\v5\odrive\ODrive Pro Assembly\Extruded_43_1.ipt
- C:\work\openworkout\digital_weight_device\cad\v5\odrive\ODrive Pro Assembly\Open CASCADE STEP translator 6.8 23.2.1_12.ipt
- C:\work\openworkout\digital_weight_device\cad\v5\odrive\ODrive Pro Assembly\Open CASCADE STEP translator 6.8 1.2.1_3.ipt
- C:\work\openworkout\digital_weight_device\cad\v5\odrive\ODrive Pro Assembly\Extruded_22_3.ipt
- C:\work\openworkout\digital_weight_device\cad\v5\odrive\ODrive Pro Assembly\Extruded_59.ipt
- C:\work\openworkout\digital_weight_device\cad\v5\odrive\ODrive Pro Assembly\Extruded_65.ipt
- C:\work\openworkout\digital_weight_device\cad\v5\odrive\ODrive Pro Assembly\Extruded_39_1.ipt
- C:\work\openworkout\digital_weight_device\cad\v5\odrive\ODrive Pro Assembly\Extruded_40_2.ipt
- C:\work\openworkout\digital_weight_device\cad\v5\odrive\ODrive Pro Assembly\Open CASCADE STEP translator 6.8 26.4.1.ipt
- C:\work\openworkout\digital_weight_device\cad\v5\odrive\ODrive Pro Assembly\FDMS86300DC rev A_1.ipt
- C:\work\openworkout\digital_weight_device\cad\v5\odrive\ODrive Pro Assembly\Extruded_14_6.ipt
- C:\work\openworkout\digital_weight_device\cad\v5\odrive\ODrive Pro Assembly\Extruded_13_6.ipt
- C:\work\openworkout\digital_weight_device\cad\v5\odrive\ODrive Pro Assembly\Extruded_29_4.ipt
- C:\work\openworkout\digital_weight_device\cad\v5\odrive\ODrive Pro Assembly\Mid_Body_4_2.ipt
- C:\work\openworkout\digital_weight_device\cad\v5\odrive\ODrive Pro Assembly\Open CASCADE STEP translator 6.8 23.2.1_5.ipt
- C:\work\openworkout\digital_weight_device\cad\v5\odrive\ODrive Pro Assembly\Extruded_12_8.ipt
- C:\work\openworkout\digital_weight_device\cad\v5\odrive\ODrive Pro Assembly\Extruded_7_5.ipt
- C:\work\openworkout\digital_weight_device\cad\v5\odrive\ODrive Pro Assembly\___________10 SIZE CODE G_2.ipt
- C:\work\openworkout\digital_weight_device\cad\v5\odrive\ODrive Pro Assembly\Leader_27.ipt
- C:\work\openworkout\digital_weight_device\cad\v5\odrive\ODrive Pro Assembly\Extruded_20_2.ipt
- C:\work\openworkout\digital_weight_device\cad\v5\odrive\ODrive Pro Assembly\Mid_Body_7.ipt
- C:\work\openworkout\digital_weight_device\cad\v5\odrive\ODrive Pro Assembly\Extruded_10_7.ipt
- C:\work\openworkout\digital_weight_device\cad\v5\odrive\ODrive Pro Assembly\Extruded_14_7.ipt
- C:\work\openworkout\digital_weight_device\cad\v5\odrive\ODrive Pro Assembly\Mark_6_1.ipt
- C:\work\openworkout\digital_weight_device\cad\v5\odrive\ODrive Pro Assembly\Extruded_41_2.ipt
- C:\work\openworkout\digital_weight_device\cad\v5\odrive\ODrive Pro Assembly\Open CASCADE STEP translator 6.8 18.2.1_1_1.ipt
- C:\work\openworkout\digital_weight_device\cad\v5\odrive\ODrive Pro Assembly\Mark_2_3.ipt
- C:\work\openworkout\digital_weight_device\cad\v5\odrive\ODrive Pro Assembly\Mid_Body_1_3.ipt
- C:\work\openworkout\digital_weight_device\cad\v5\odrive\ODrive Pro Assembly\Extruded_47_1.ipt
- C:\work\openworkout\digital_weight_device\cad\v5\odrive\ODrive Pro Assembly\Extruded_11_4.ipt
- C:\work\openworkout\digital_weight_device\cad\v5\odrive\ODrive Pro Assembly\Cylinder_8_1.ipt
- C:\work\openworkout\digital_weight_device\cad\v5\odrive\ODrive Pro Assembly\Extruded_34_3.ipt
- C:\work\openworkout\digital_weight_device\cad\v5\odrive\ODrive Pro Assembly\Extruded_14_8.ipt
- C:\work\openworkout\digital_weight_device\cad\v5\odrive\ODrive Pro Assembly\Leader_5_2.ipt
- C:\work\openworkout\digital_weight_device\cad\v5\odrive\ODrive Pro Assembly\Open CASCADE STEP translator 6.8 2.1.1_6.ipt
- C:\work\openworkout\digital_weight_device\cad\v5\odrive\ODrive Pro Assembly\Leader_13.ipt
- C:\work\openworkout\digital_weight_device\cad\v5\odrive\ODrive Pro Assembly\Leader_6.ipt
- C:\work\openworkout\digital_weight_device\cad\v5\odrive\ODrive Pro Assembly\Extruded_21_2.ipt
- C:\work\openworkout\digital_weight_device\cad\v5\odrive\ODrive Pro Assembly\SOT23-6.ipt
- C:\work\openworkout\digital_weight_device\cad\v5\odrive\ODrive Pro Assembly\Extruded_9_6.ipt
- C:\work\openworkout\digital_weight_device\cad\v5\odrive\ODrive Pro Assembly\Open CASCADE STEP translator 6.8 2.1.2_1.ipt
- C:\work\openworkout\digital_weight_device\cad\v5\odrive\ODrive Pro Assembly\Extruded_9_7.ipt
- C:\work\openworkout\digital_weight_device\cad\v5\odrive\ODrive Pro Assembly\Extruded_1_10.ipt
- C:\work\openworkout\digital_weight_device\cad\v5\odrive\ODrive Pro Assembly\Extruded_8_6.ipt
- C:\work\openworkout\digital_weight_device\cad\v5\odrive\ODrive Pro Assembly\Extruded_7_6.ipt
- C:\work\openworkout\digital_weight_device\cad\v5\odrive\ODrive Pro Assembly\Extruded_4_5.ipt
- C:\work\openworkout\digital_weight_device\cad\v5\odrive\ODrive Pro Assembly\Open CASCADE STEP translator 6.8 2.1.2_3.ipt
- C:\work\openworkout\digital_weight_device\cad\v5\odrive\ODrive Pro Assembly\Open CASCADE STEP translator 6.8 43.4.1_9.ipt
- C:\work\openworkout\digital_weight_device\cad\v5\odrive\ODrive Pro Assembly\Open CASCADE STEP translator 6.8 43.4.1_2.ipt
- C:\work\openworkout\digital_weight_device\cad\v5\odrive\ODrive Pro Assembly\Open CASCADE STEP translator 6.8 1.2.1_5.ipt
- C:\work\openworkout\digital_weight_device\cad\v5\odrive\ODrive Pro Assembly\Extruded_11_5.ipt
- C:\work\openworkout\digital_weight_device\cad\v5\odrive\ODrive Pro Assembly\Extruded_53.ipt
- C:\work\openworkout\digital_weight_device\cad\v5\odrive\ODrive Pro Assembly\Extruded_2_5.ipt
- C:\work\openworkout\digital_weight_device\cad\v5\odrive\ODrive Pro Assembly\Cylinder_11_1.ipt
- C:\work\openworkout\digital_weight_device\cad\v5\odrive\ODrive Pro Assembly\Extruded_2_6.ipt
- C:\work\openworkout\digital_weight_device\cad\v5\odrive\ODrive Pro Assembly\Extruded_3_9.ipt
- C:\work\openworkout\digital_weight_device\cad\v5\odrive\ODrive Pro Assembly\Extruded_56.ipt
- C:\work\openworkout\digital_weight_device\cad\v5\odrive\ODrive Pro Assembly\Extruded_2_7.ipt
- C:\work\openworkout\digital_weight_device\cad\v5\odrive\ODrive Pro Assembly\Extruded_5_8.ipt
- C:\work\openworkout\digital_weight_device\cad\v5\odrive\ODrive Pro Assembly\Extruded_7_7.ipt
- C:\work\openworkout\digital_weight_device\cad\v5\odrive\ODrive Pro Assembly\Extruded_28_3.ipt
- C:\work\openworkout\digital_weight_device\cad\v5\odrive\ODrive Pro Assembly\Extruded_11_6.ipt
- C:\work\openworkout\digital_weight_device\cad\v5\odrive\ODrive Pro Assembly\Extruded_60.ipt
- C:\work\openworkout\digital_weight_device\cad\v5\odrive\ODrive Pro Assembly\Extruded_32_2.ipt
- C:\work\openworkout\digital_weight_device\cad\v5\odrive\ODrive Pro Assembly\Extruded_25_3.ipt
- C:\work\openworkout\digital_weight_device\cad\v5\odrive\ODrive Pro Assembly\Mark_3_2.ipt
- C:\work\openworkout\digital_weight_device\cad\v5\odrive\ODrive Pro Assembly\Mid_Body_2_2.ipt
- C:\work\openworkout\digital_weight_device\cad\v5\odrive\ODrive Pro Assembly\Open CASCADE STEP translator 6.8 8.1.ipt
- C:\work\openworkout\digital_weight_device\cad\v5\odrive\ODrive Pro Assembly\Open CASCADE STEP translator 6.8 1.2.1_7.ipt
- C:\work\openworkout\digital_weight_device\cad\v5\odrive\ODrive Pro Assembly\RES 0603 (1608 metric)_17.ipt
- C:\work\openworkout\digital_weight_device\cad\v5\odrive\ODrive Pro Assembly\RES 0603 (1608 metric)_6.ipt
- C:\work\openworkout\digital_weight_device\cad\v5\odrive\ODrive Pro Assembly\RES 0603 (1608 metric)_14.ipt
- C:\work\openworkout\digital_weight_device\cad\v5\odrive\ODrive Pro Assembly\Extruded_20_3.ipt
- C:\work\openworkout\digital_weight_device\cad\v5\odrive\ODrive Pro Assembly\Leader_4_1.ipt
- C:\work\openworkout\digital_weight_device\cad\v5\odrive\ODrive Pro Assembly\Extruded_57.ipt
- C:\work\openworkout\digital_weight_device\cad\v5\odrive\ODrive Pro Assembly\Open CASCADE STEP translator 6.8 26.4.1_2.ipt
- C:\work\openworkout\digital_weight_device\cad\v5\odrive\ODrive Pro Assembly\Mid_Body_8.ipt
- C:\work\openworkout\digital_weight_device\cad\v5\odrive\ODrive Pro Assembly\FDMS86300DC rev A_10.ipt
- C:\work\openworkout\digital_weight_device\cad\v5\odrive\ODrive Pro Assembly\FDMS86300DC rev A_3.ipt
- C:\work\openworkout\digital_weight_device\cad\v5\odrive\ODrive Pro Assembly\Extruded_22_4.ipt
- C:\work\openworkout\digital_weight_device\cad\v5\odrive\ODrive Pro Assembly\Mark_1_3.ipt
- C:\work\openworkout\digital_weight_device\cad\v5\odrive\ODrive Pro Assembly\Mid_Body_9.ipt
- C:\work\openworkout\digital_weight_device\cad\v5\odrive\ODrive Pro Assembly\Extruded_13_7.ipt
- C:\work\openworkout\digital_weight_device\cad\v5\odrive\ODrive Pro Assembly\Extruded_29_5.ipt
- C:\work\openworkout\digital_weight_device\cad\v5\odrive\ODrive Pro Assembly\Open CASCADE STEP translator 6.8 23.2.1_1_2.ipt
- C:\work\openworkout\digital_weight_device\cad\v5\odrive\ODrive Pro Assembly\Extruded_30_3.ipt
- C:\work\openworkout\digital_weight_device\cad\v5\odrive\ODrive Pro Assembly\Extruded_32_3.ipt
- C:\work\openworkout\digital_weight_device\cad\v5\odrive\ODrive Pro Assembly\Cylinder_6_1.ipt
- C:\work\openworkout\digital_weight_device\cad\v5\odrive\ODrive Pro Assembly\Extruded_18_2.ipt
- C:\work\openworkout\digital_weight_device\cad\v5\odrive\ODrive Pro Assembly\Open CASCADE STEP translator 6.8 23.2.1_9_2.ipt
- C:\work\openworkout\digital_weight_device\cad\v5\odrive\ODrive Pro Assembly\Extruded_28_4.ipt
- C:\work\openworkout\digital_weight_device\cad\v5\odrive\ODrive Pro Assembly\Mid_Body_4_3.ipt
- C:\work\openworkout\digital_weight_device\cad\v5\odrive\ODrive Pro Assembly\Extruded_36_1.ipt
- C:\work\openworkout\digital_weight_device\cad\v5\odrive\ODrive Pro Assembly\Extruded_39_2.ipt
- C:\work\openworkout\digital_weight_device\cad\v5\odrive\ODrive Pro Assembly\Extruded_12_9.ipt
- C:\work\openworkout\digital_weight_device\cad\v5\odrive\ODrive Pro Assembly\Extruded_6_8.ipt
- C:\work\openworkout\digital_weight_device\cad\v5\odrive\ODrive Pro Assembly\______10 SIZE CODE G.ipt
- C:\work\openworkout\digital_weight_device\cad\v5\odrive\ODrive Pro Assembly\Extruded_16_4.ipt
- C:\work\openworkout\digital_weight_device\cad\v5\odrive\ODrive Pro Assembly\________10 SIZE CODE G_5.ipt
- C:\work\openworkout\digital_weight_device\cad\v5\odrive\ODrive Pro Assembly\________10 SIZE CODE G_2.ipt
- C:\work\openworkout\digital_weight_device\cad\v5\odrive\ODrive Pro Assembly\Extruded_7_8.ipt
- C:\work\openworkout\digital_weight_device\cad\v5\odrive\ODrive Pro Assembly\Mark_3_3.ipt
- C:\work\openworkout\digital_weight_device\cad\v5\odrive\ODrive Pro Assembly\Extruded_7_9.ipt
- C:\work\openworkout\digital_weight_device\cad\v5\odrive\ODrive Pro Assembly\Extruded_18_3.ipt
- C:\work\openworkout\digital_weight_device\cad\v5\odrive\ODrive Pro Assembly\Extruded_10_8.ipt
- C:\work\openworkout\digital_weight_device\cad\v5\odrive\ODrive Pro Assembly\Extruded_3_10.ipt
- C:\work\openworkout\digital_weight_device\cad\v5\odrive\ODrive Pro Assembly\Open CASCADE STEP translator 6.8 23.2.1_7.ipt
- C:\work\openworkout\digital_weight_device\cad\v5\odrive\ODrive Pro Assembly\Open CASCADE STEP translator 6.8 23.2.1_1_3.ipt
- C:\work\openworkout\digital_weight_device\cad\v5\odrive\ODrive Pro Assembly\Extruded_2_8.ipt
- C:\work\openworkout\digital_weight_device\cad\v5\odrive\ODrive Pro Assembly\Extruded_21_3.ipt
- C:\work\openworkout\digital_weight_device\cad\v5\odrive\ODrive Pro Assembly\Extruded_5_9.ipt
- C:\work\openworkout\digital_weight_device\cad\v5\odrive\ODrive Pro Assembly\Open CASCADE STEP translator 6.8 2.2.1_1_1.ipt
- C:\work\openworkout\digital_weight_device\cad\v5\odrive\ODrive Pro Assembly\Cylinder_10_1.ipt
- C:\work\openworkout\digital_weight_device\cad\v5\odrive\ODrive Pro Assembly\Mid_Body_2_3.ipt
- C:\work\openworkout\digital_weight_device\cad\v5\odrive\ODrive Pro Assembly\Open CASCADE STEP translator 7.5 6.64.1.1.ipt
- C:\work\openworkout\digital_weight_device\cad\v5\odrive\ODrive Pro Assembly\Extruded_58.ipt
- C:\work\openworkout\digital_weight_device\cad\v5\odrive\ODrive Pro Assembly\Extruded_6_9.ipt
- C:\work\openworkout\digital_weight_device\cad\v5\odrive\ODrive Pro Assembly\Open CASCADE STEP translator 6.8 43.4.1.ipt
- C:\work\openworkout\digital_weight_device\cad\v5\odrive\ODrive Pro Assembly\Leader_20.ipt
- C:\work\openworkout\digital_weight_device\cad\v5\odrive\ODrive Pro Assembly\Extruded_15_7.ipt
- C:\work\openworkout\digital_weight_device\cad\v5\odrive\ODrive Pro Assembly\RES 0603 (1608 metric)_1.ipt
- C:\work\openworkout\digital_weight_device\cad\v5\odrive\ODrive Pro Assembly\Extruded_64.ipt
- C:\work\openworkout\digital_weight_device\cad\v5\odrive\ODrive Pro Assembly\Leader_29.ipt